# Autodesk Inventor assembly: axis4
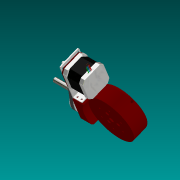
[picture p0: Inventor's stored thumbnail of the model, 180x180]
Saved by Autodesk Inventor 2020.3 (Build 243373000, 373)
## iProperties
Created: 2020-05-24
Part Number: axis4
Document SubType Name: Assembly
Designer: Svend
Author: Svend
## Documents named in this file (11)
- C:\Users\Svend\OneDrive\Documents\GitHub\BeerMinder\3D-model\axis4\axis4.iam
- C:\Users\Svend\OneDrive\Documents\GitHub\BeerMinder\3D-model\Base (Axis 1)\as4mount.ipt
- C:\Users\Svend\OneDrive\Documents\GitHub\BeerMinder\3D-model\pulleys\GT2 Timing Pulley 60T - 8mm as.ipt
- C:\Users\Svend\OneDrive\Documents\GitHub\BeerMinder\3D-model\stepper motors\42BYG Stepper Motor.ipt
- C:\Users\Svend\OneDrive\Documents\GitHub\BeerMinder\3D-model\pulleys\GT2 Pulley 16T - 5mm as.ipt
- C:\Users\Svend\OneDrive\Documents\GitHub\BeerMinder\3D-model\pulleys\Tandriem16naar60T.ipt
- C:\Users\Svend\OneDrive\Documents\GitHub\BeerMinder\3D-model\Base (Axis 1)\asArm2.ipt
- C:\Users\Svend\OneDrive\Documents\GitHub\BeerMinder\3D-model\bearings\Ball Bearing 608ZZ.ipt
- C:\Users\Svend\OneDrive\Documents\GitHub\BeerMinder\3D-model\axis4\asmountAs4.ipt
- C:\Users\Svend\OneDrive\Documents\GitHub\BeerMinder\3D-model\axis4\steppermount.ipt
- C:\Users\Svend\OneDrive\Documents\GitHub\BeerMinder\3D-model\axis4\stepperspacer.ipt
## Components (10 placed, 10 different names)
1. as4mount:1 — Mate:3, Mate:4, Mate:5, Mate:9, Angle:1, Mate:10, Flush:1, Flush:2, Mate:15, Angle:2, Flush:8, Mate:16, Mate:17, Mate:18
2. GT2 Timing Pulley 60T - 8mm as:1 — Mate:5, Mate:6, Mate:7, Mate:8, Mate:14
3. 42BYG Stepper Motor:1 — Mate:13, Angle:2, Flush:8, Mate:19, Mate:20, Mate:21
4. GT2 Pulley 16T - 5mm as:1 — Mate:11, Mate:12, Mate:13
5. Tandriem16naar60T:1 — Mate:7, Mate:8, Mate:11, Mate:12
6. asArm2:1 — Mate:14, Mate:15
7. Ball Bearing 608ZZ:1 — Mate:3, Mate:4, Mate:6
8. asmountAs4:1 — Mate:9, Angle:1, Mate:10, Flush:1, Flush:2
9. steppermount:1 — Mate:16, Mate:17, Mate:18, Mate:22
10. stepperspacer:1 — Mate:19, Mate:20, Mate:21, Mate:22
## Relationships (25: Mate 20, Flush 3, Angle 2)
- Mate:3: as4mount:1 ↔ Ball Bearing 608ZZ:1
- Mate:4: as4mount:1 ↔ Ball Bearing 608ZZ:1
- Mate:5: as4mount:1 ↔ GT2 Timing Pulley 60T - 8mm as:1
- Mate:6: GT2 Timing Pulley 60T - 8mm as:1 ↔ Ball Bearing 608ZZ:1
- Mate:7: GT2 Timing Pulley 60T - 8mm as:1 ↔ Tandriem16naar60T:1
- Mate:8 (0.5 mm): GT2 Timing Pulley 60T - 8mm as:1 ↔ Tandriem16naar60T:1
- Mate:9: as4mount:1 ↔ asmountAs4:1
- Angle:1 (108 deg): as4mount:1 ↔ asmountAs4:1
- Mate:10: as4mount:1 ↔ asmountAs4:1
- Flush:1: as4mount:1 ↔ asmountAs4:1
- Flush:2: as4mount:1 ↔ asmountAs4:1
- Mate:11: GT2 Pulley 16T - 5mm as:1 ↔ Tandriem16naar60T:1
- Mate:12 (0.5 mm): GT2 Pulley 16T - 5mm as:1 ↔ Tandriem16naar60T:1
- Mate:13: 42BYG Stepper Motor:1 ↔ GT2 Pulley 16T - 5mm as:1
- Mate:14: GT2 Timing Pulley 60T - 8mm as:1 ↔ asArm2:1
- Mate:15: as4mount:1 ↔ asArm2:1
- Angle:2 (180 deg): as4mount:1 ↔ 42BYG Stepper Motor:1
- Flush:8: as4mount:1 ↔ 42BYG Stepper Motor:1
- Mate:16: as4mount:1 ↔ steppermount:1
- Mate:17: as4mount:1 ↔ steppermount:1
- Mate:18: as4mount:1 ↔ steppermount:1
- Mate:19: 42BYG Stepper Motor:1 ↔ stepperspacer:1
- Mate:20: 42BYG Stepper Motor:1 ↔ stepperspacer:1
- Mate:21: 42BYG Stepper Motor:1 ↔ stepperspacer:1
- Mate:22: steppermount:1 ↔ stepperspacer:1
